# Autodesk Inventor assembly: Assembly
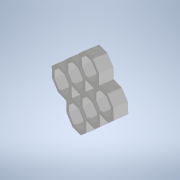
[picture p0: Inventor's stored thumbnail of the model, 180x180]
Saved by Autodesk Inventor 2020 (Build 240168000, 168)
## iProperties
Created: 2020-06-16
Part Number: Assembly
Document SubType Name: Assembly
Designer: user
Author: user
## Documents named in this file (2)
- C:\Users\user\Documents\Github\3D_Designs\MagicTokenHolder\Assembly.iam
- C:\Users\user\Documents\Github\3D_Designs\MagicTokenHolder\TokenHolderSingle.ipt
## Components (6 placed, 1 different names)
1. TokenHolderSingle:1 — Mate:1, Flush:1, Flush:2, Flush:3, Flush:4, Mate:2, Flush:5, Flush:6, Flush:7, Flush:8, Mate:5, Flush:19, Flush:20, Flush:21
2. TokenHolderSingle:2 — Mate:1, Flush:1, Flush:2, Flush:3, Flush:4, Mate:3, Flush:9, Flush:10
3. TokenHolderSingle:3 — Mate:2, Flush:5, Flush:6, Flush:7, Flush:8, Flush:11, Flush:12, Flush:17, Flush:18
4. TokenHolderSingle:4 — Mate:3, Flush:9, Flush:10, Flush:11, Flush:12
5. TokenHolderSingle:5 — Mate:5, Flush:19, Flush:20, Flush:21
6. TokenHolderSingle:6 — Flush:17, Flush:18
## Relationships (26: Flush 21, Mate 5)
- Mate:1: TokenHolderSingle:1 ↔ TokenHolderSingle:2
- Flush:1: TokenHolderSingle:1 ↔ TokenHolderSingle:2
- Flush:2: TokenHolderSingle:1 ↔ TokenHolderSingle:2
- Flush:3: TokenHolderSingle:1 ↔ TokenHolderSingle:2
- Flush:4: TokenHolderSingle:1 ↔ TokenHolderSingle:2
- Mate:2: TokenHolderSingle:1 ↔ TokenHolderSingle:3
- Flush:5: TokenHolderSingle:1 ↔ TokenHolderSingle:3
- Flush:6: TokenHolderSingle:1 ↔ TokenHolderSingle:3
- Flush:7: TokenHolderSingle:1 ↔ TokenHolderSingle:3
- Flush:8: TokenHolderSingle:1 ↔ TokenHolderSingle:3
- Mate:3: TokenHolderSingle:2 ↔ TokenHolderSingle:4
- Flush:9: TokenHolderSingle:2 ↔ TokenHolderSingle:4
- Flush:10: TokenHolderSingle:2 ↔ TokenHolderSingle:4
- Flush:11: TokenHolderSingle:3 ↔ TokenHolderSingle:4
- Flush:12: TokenHolderSingle:3 ↔ TokenHolderSingle:4
- [Mate]: TokenHolderSingle:5 ↔ TokenHolderSingle:6
- [Flush]: TokenHolderSingle:5 ↔ TokenHolderSingle:6
- [Flush]: TokenHolderSingle:5 ↔ TokenHolderSingle:6
- [Flush]: TokenHolderSingle:5 ↔ TokenHolderSingle:6
- [Flush]: TokenHolderSingle:5 ↔ TokenHolderSingle:6
- Mate:5: TokenHolderSingle:1 ↔ TokenHolderSingle:5
- Flush:17: TokenHolderSingle:3 ↔ TokenHolderSingle:6
- Flush:18: TokenHolderSingle:3 ↔ TokenHolderSingle:6
- Flush:19: TokenHolderSingle:1 ↔ TokenHolderSingle:5
- Flush:20: TokenHolderSingle:1 ↔ TokenHolderSingle:5
- Flush:21: TokenHolderSingle:1 ↔ TokenHolderSingle:5
## Named parameters: d17_d5 = 0 mm, d18_d6 = 0 mm, d19_d7 = 0 mm, d20_d8 = 0 mm, d21_d9 = 0 mm
